# Autodesk Inventor assembly: essemble
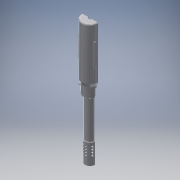
[picture p0: Inventor's stored thumbnail of the model, 180x180]
Saved by Autodesk Inventor 2019 (Build 230136000, 136)
## iProperties
Created: 2018-04-25
Part Number: essemble
Material: Générique
Document SubType Name: Assembly
Designer: Theo
Author: Theo
## Documents named in this file (5)
- D:\dev\projects\canon-ace\ACE 20 B\essemble.iam
- D:\dev\projects\canon-ace\ACE 20 B\reservoir.ipt
- D:\dev\projects\canon-ace\ACE 20 B\canon.ipt
- D:\dev\projects\canon-ace\ACE 20 B\douille.ipt
- D:\dev\projects\canon-ace\ACE 20 B\joint.ipt
## Components (4 placed, 4 different names)
1. reservoir:1 — Placage:1, Placage:8, Placage:9, Placage:11
2. canon:1 — Placage:1, Placage:10, Placage:12, Placage:13
3. douille:1 — Placage:9, Placage:10, Placage:11, Placage:12, Placage:13
4. joint:1 — Placage:8
## Relationships (7: Mate 7)
- Placage:1 [Mate]: reservoir:1 ↔ canon:1
- Placage:8 [Mate]: reservoir:1 ↔ joint:1
- Placage:9 [Mate]: reservoir:1 ↔ douille:1
- Placage:10 [Mate]: canon:1 ↔ douille:1
- Placage:11 [Mate]: reservoir:1 ↔ douille:1
- Placage:12 [Mate]: canon:1 ↔ douille:1
- Placage:13 [Mate]: canon:1 ↔ douille:1
